# Autodesk Inventor assembly: korp
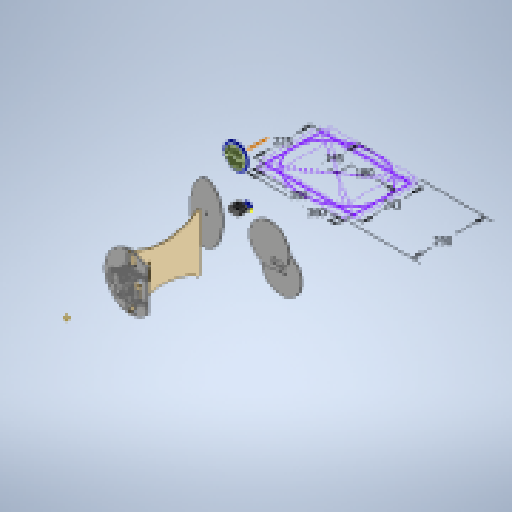
[picture p0: Inventor's stored thumbnail of the model, 512x512]
Saved by Autodesk Inventor 2023.1 (Build 271208000, 208)
## iProperties
Created: 2023-03-13
Part Number: korp
Document SubType Name: Assembly
Designer: User
Author: User
## Documents named in this file (17)
- C:\Users\DELL\reposGitHub\Cheburashka\Cheburashka_construction\korpus\korp.iam
- C:\Users\DELL\reposGitHub\Cheburashka\Cheburashka_construction\korpus\нижний эллипс тела.ipt
- C:\Users\DELL\reposGitHub\Cheburashka\Cheburashka_construction\korpus\грань тела.ipt
- C:\Users\DELL\reposGitHub\Cheburashka\Cheburashka_construction\korpus\верхний эллипс туловища.ipt
- C:\Users\DELL\reposGitHub\Cheburashka\Cheburashka_construction\korpus\нижний эллипс головы.ipt
- C:\Users\DELL\reposGitHub\Cheburashka\Cheburashka_construction\korpus\Servo.ipt
- C:\Users\DELL\reposGitHub\Cheburashka\Cheburashka_construction\korpus\Pitsco Education-739028.ipt
- C:\Users\DELL\reposGitHub\Cheburashka\Cheburashka_construction\korpus\Pitsco Education-739085.ipt
- C:\Users\DELL\reposGitHub\Cheburashka\Cheburashka_construction\korpus\трубка.ipt
- C:\Users\DELL\reposGitHub\Cheburashka\Cheburashka_construction\korpus\Prostavka.ipt
- C:\Users\DELL\reposGitHub\Cheburashka\Cheburashka_construction\korpus\лицо1.ipt
- C:\Users\DELL\reposGitHub\Cheburashka\Cheburashka_construction\korpus\att_pin.ipt
- C:\Users\DELL\reposGitHub\Cheburashka\Cheburashka_construction\platform\print\Деталь1.ipt
- C:\Users\DELL\reposGitHub\Cheburashka\Cheburashka_construction\platform\KRAVT_holder_2 (1).ipt
- C:\Users\DELL\reposGitHub\Cheburashka\Cheburashka_construction\platform\стойка.ipt
- C:\Users\DELL\reposGitHub\Cheburashka\Cheburashka_construction\platform\Raspberry Pi 4 Model B.iam
- C:\Users\DELL\reposGitHub\Cheburashka\Cheburashka_construction\korpus\arduino MEGA2650.iam
## Components (20 placed, 16 different names)
1. нижний эллипс тела:1 — Совмещение:100
2. верхний эллипс туловища:1
3. грань тела:1 — Совмещение:101, Совмещение:102, Совмещение:103, Совмещение:104, Совмещение:105, Совмещение:106
4. нижний эллипс головы:1 — Совмещение:73
5. Pitsco Education-739028:1 — Совмещение:99
6. Pitsco Education-739085:1 — Совмещение:68, Совмещение:75, Совмещение:80
7. трубка:1 — Совмещение:68, Совмещение:74, Совмещение:81
8. Servo:4 — Совмещение:97, Совмещение:98
9. Prostavka:1 — Совмещение:73, Совмещение:74, Совмещение:75
10. Prostavka:2 — Совмещение:80, Совмещение:81, Заподлицо:16
11. лицо1:1 — Заподлицо:16, Заподлицо:17
12. att_pin:1 — Совмещение:97, Совмещение:98, Совмещение:99
13. Деталь1:1 — Заподлицо:17
14. KRAVT_holder_2 (1):1 — Совмещение:100, Совмещение:101
15. стойка:1 — Совмещение:102, Совмещение:103
16. стойка:2 — Совмещение:106
17. стойка:3 — Совмещение:104
18. стойка:4 — Совмещение:105
19. Raspberry Pi 4 Model B:1 [sub-assembly]
20. arduino MEGA2650:1 [sub-assembly]
## Relationships (18: Mate 16, Flush 2)
- Совмещение:68 [Mate]: Pitsco Education-739085:1 ↔ трубка:1
- Совмещение:73 [Mate]: нижний эллипс головы:1 ↔ Prostavka:1
- Совмещение:74 [Mate]: трубка:1 ↔ Prostavka:1
- Совмещение:75 [Mate]: Pitsco Education-739085:1 ↔ Prostavka:1
- Совмещение:80 [Mate]: Pitsco Education-739085:1 ↔ Prostavka:2
- Совмещение:81 [Mate]: трубка:1 ↔ Prostavka:2
- Заподлицо:16 [Flush]: Prostavka:2 ↔ лицо1:1
- Совмещение:97 [Mate]: Servo:4 ↔ att_pin:1
- Совмещение:98 [Mate]: Servo:4 ↔ att_pin:1
- Совмещение:99 [Mate]: Pitsco Education-739028:1 ↔ att_pin:1
- Заподлицо:17 [Flush]: лицо1:1 ↔ Деталь1:1
- Совмещение:100 [Mate]: нижний эллипс тела:1 ↔ KRAVT_holder_2 (1):1
- Совмещение:101 [Mate] (56.5 mm): грань тела:1 ↔ KRAVT_holder_2 (1):1
- Совмещение:102 [Mate]: грань тела:1 ↔ стойка:1
- Совмещение:103 [Mate]: грань тела:1 ↔ стойка:1
- Совмещение:104 [Mate]: грань тела:1 ↔ стойка:3
- Совмещение:105 [Mate]: грань тела:1 ↔ стойка:4
- Совмещение:106 [Mate]: грань тела:1 ↔ стойка:2
